# Autodesk Inventor assembly: outer
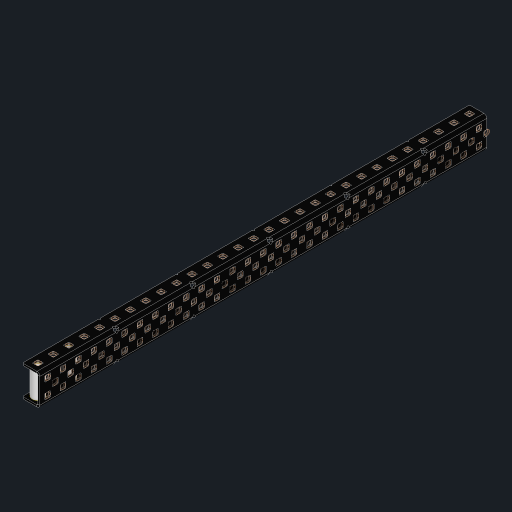
[picture p0: Inventor's stored thumbnail of the model, 512x512]
Saved by Autodesk Inventor 2024 (Build 280153000, 153)
## iProperties
Created: 2024-05-12
Part Number: outer
Document SubType Name: Assembly
Designer: Averey Ku
Author: Averey Ku
## Documents named in this file (4)
- D:\vex_robotics\hardware\cad\kdot\chassis\drivebay\outer.iam
- D:\vex_robotics\hardware\cad\VEX-CAD-Inventor-1.41\Structure\C Channel\Aluminum 1x2x1\Alu C 1x2x1x29.ipt
- D:\vex_robotics\hardware\cad\VEX-CAD-Inventor-1.41\Motion\Shaft LS\Bearing Flat Low Profile.ipt
- D:\vex_robotics\hardware\cad\hardware\.375 OD Aluminum Spacer 0.875.ipt
## Components (10 placed, 3 different names)
1. Alu C 1x2x1x29:2 — Insert:2, Mate:2, Insert:3, Mate:3, Insert:4, Mate:4, Insert:5, Mate:5, Insert:6, Mate:6, Insert:7, Mate:7, Insert:8, Mate:8, Insert:9, Insert:10
2. Bearing Flat Low Profile:1 — Insert:8, Mate:8
3. Bearing Flat Low Profile:2 — Insert:2, Mate:2
4. Bearing Flat Low Profile:3 — Insert:3, Mate:3
5. Bearing Flat Low Profile:4 — Insert:4, Mate:4
6. Bearing Flat Low Profile:5 — Insert:5, Mate:5
7. Bearing Flat Low Profile:6 — Insert:6, Mate:6
8. Bearing Flat Low Profile:7 — Insert:7, Mate:7
9. .375 OD Aluminum Spacer 0.875:1 — Insert:10
10. .375 OD Aluminum Spacer 0.875:2 — Insert:9
## Relationships (16: Insert 9, Mate 7)
- Insert:2: Alu C 1x2x1x29:2 ↔ Bearing Flat Low Profile:2
- Mate:2: Alu C 1x2x1x29:2 ↔ Bearing Flat Low Profile:2
- Insert:3: Alu C 1x2x1x29:2 ↔ Bearing Flat Low Profile:3
- Mate:3: Alu C 1x2x1x29:2 ↔ Bearing Flat Low Profile:3
- Insert:4: Alu C 1x2x1x29:2 ↔ Bearing Flat Low Profile:4
- Mate:4: Alu C 1x2x1x29:2 ↔ Bearing Flat Low Profile:4
- Insert:5: Alu C 1x2x1x29:2 ↔ Bearing Flat Low Profile:5
- Mate:5: Alu C 1x2x1x29:2 ↔ Bearing Flat Low Profile:5
- Insert:6: Alu C 1x2x1x29:2 ↔ Bearing Flat Low Profile:6
- Mate:6: Alu C 1x2x1x29:2 ↔ Bearing Flat Low Profile:6
- Insert:7: Alu C 1x2x1x29:2 ↔ Bearing Flat Low Profile:7
- Mate:7: Alu C 1x2x1x29:2 ↔ Bearing Flat Low Profile:7
- Insert:8: Alu C 1x2x1x29:2 ↔ Bearing Flat Low Profile:1
- Mate:8: Alu C 1x2x1x29:2 ↔ Bearing Flat Low Profile:1
- Insert:9: Alu C 1x2x1x29:2 ↔ .375 OD Aluminum Spacer 0.875:2
- Insert:10: Alu C 1x2x1x29:2 ↔ .375 OD Aluminum Spacer 0.875:1
